# Autodesk Inventor assembly: AliCe_Motor_l
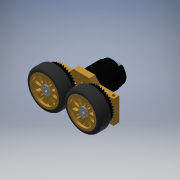
[picture p0: Inventor's stored thumbnail of the model, 180x180]
Saved by Autodesk Inventor 2016 (Build 200138000, 138)
## iProperties
Created: 2016-12-01
Part Number: AliCe_Motor_l
Material: 一般
Document SubType Name: Assembly
Designer: KOTA-NPC2
Author: KOTA-NPC2
## Documents named in this file (10)
- C:\Users\B4_Ohno\Dropbox\AliCe\MicroMouse2016\AliCe_Motor_l.iam
- C:\Users\B4_Ohno\Dropbox\AliCe\MicroMouse2016\1717.ipt
- C:\Users\B4_Ohno\Dropbox\AliCe\MicroMouse2016\AliCe_Motor\デザイン アクセラレータ\平歯車14.ipt
- C:\Users\B4_Ohno\Dropbox\AliCe\MicroMouse2016\Tire.ipt
- C:\Users\B4_Ohno\Dropbox\AliCe\MicroMouse2016\Wheel.ipt
- C:\Users\B4_Ohno\Dropbox\AliCe\MicroMouse2016\スパーギア.ipt
- C:\Users\B4_Ohno\Dropbox\AliCe\MicroMouse2016\ベアリング.ipt
- C:\Users\B4_Ohno\Dropbox\AliCe\MicroMouse2016\ナット.ipt
- C:\Users\B4_Ohno\Dropbox\AliCe\MicroMouse2016\シムリング.ipt
- C:\Users\B4_Ohno\Dropbox\AliCe\MicroMouse2016\m_mount_l.ipt
## Components (17 placed, 9 different names)
1. 1717:1 — 回転:6, リジッド:21
2. 平歯車1:1 — 回転:6
3. 平歯車2:3 — W+G:1, S+B:1
4. 平歯車2:4 — W+G:2, リジッド:17
5. Tire:2 — W+T:1
6. Wheel:2 — W+T:1, W+G:1, 回転:4
7. ベアリング:1 — S+B:1, B+S:1
8. ベアリング:4 — B+S:2, リジッド:17
9. ナット:1 — リジッド:20
10. ナット:2 — リジッド:19
11. シムリング:1 — B+S:2, 回転:5
12. シムリング:2 — B+S:1, 回転:7
13. Tire:3 — W+T:2
14. Wheel:3 — W+T:2, W+G:2, リジッド:18
15. ベアリング:5 — 回転:4
16. ベアリング:6 — リジッド:18
17. m_mount_l:1 — リジッド:19, リジッド:20, 回転:5, 回転:7, リジッド:21
## Relationships (16: WeldJoint 12, RevoluteJoint 4)
- W+T:1 [WeldJoint]: Tire:2 ↔ Wheel:2
- W+T:2 [WeldJoint]: Tire:3 ↔ Wheel:3
- W+G:1 [WeldJoint]: 平歯車2:3 ↔ Wheel:2
- W+G:2 [WeldJoint]: 平歯車2:4 ↔ Wheel:3
- S+B:1 [WeldJoint]: 平歯車2:3 ↔ ベアリング:1
- B+S:2 [WeldJoint]: ベアリング:4 ↔ シムリング:1
- B+S:1 [WeldJoint]: ベアリング:1 ↔ シムリング:2
- リジッド:17 [WeldJoint]: 平歯車2:4 ↔ ベアリング:4
- 回転:4 [RevoluteJoint]: Wheel:2 ↔ ベアリング:5
- リジッド:18 [WeldJoint]: Wheel:3 ↔ ベアリング:6
- リジッド:19 [WeldJoint]: ナット:2 ↔ m_mount_l:1
- リジッド:20 [WeldJoint]: ナット:1 ↔ m_mount_l:1
- 回転:5 [RevoluteJoint]: シムリング:1 ↔ m_mount_l:1
- 回転:6 [RevoluteJoint]: 1717:1 ↔ 平歯車1:1
- 回転:7 [RevoluteJoint]: シムリング:2 ↔ m_mount_l:1
- リジッド:21 [WeldJoint]: 1717:1 ↔ m_mount_l:1
